# Autodesk Inventor assembly: Assembly_Cube_Lens_holder_v3
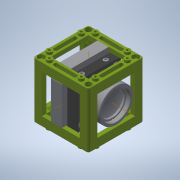
[picture p0: Inventor's stored thumbnail of the model, 180x180]
Saved by Autodesk Inventor 2022.3 (Build 263350000, 350)
## iProperties
Created: 2020-11-11
Part Number: Assembly_Cube_Lens_holder_v3
Document SubType Name: Assembly
Designer: marsikovabarbora
Author: marsikovabarbora
## Documents named in this file (5)
- G:\My Drive\ASP - M.Sc. Photonics\Practical Modules\MODULE 4 - Master Thesis\2.Experiments\Modules\8.Lens_Thorlabs_Module\Assembly_Cube_Thorlabs_Lens_Cage_v3.iam
- G:\My Drive\ASP - M.Sc. Photonics\Practical Modules\MODULE 4 - Master Thesis\2.Experiments\Modules\2.Base_Cube\Base_Cube_IM\Assembly_Cube_empty_IM_v3.iam
- G:\My Drive\ASP - M.Sc. Photonics\Practical Modules\MODULE 4 - Master Thesis\2.Experiments\Modules\8.Lens_Thorlabs_Module\00_Thorlabs_Cage_CP33_M.ipt
- G:\My Drive\ASP - M.Sc. Photonics\Practical Modules\MODULE 4 - Master Thesis\2.Experiments\Modules\8.Lens_Thorlabs_Module\20_Cube_Insert_Thorlabs_Pins.ipt
- G:\My Drive\ASP - M.Sc. Photonics\Practical Modules\MODULE 4 - Master Thesis\2.Experiments\Modules\8.Lens_Thorlabs_Module\00_THORLABS_AC254-050-A-ML-Step.ipt
## Components (4 placed, 4 different names)
1. Assembly_Cube_empty_IM_v3:1 [sub-assembly] — Mate:1, Mate:2, Mate:3, Passend:4, Passend:5
2. 00_Thorlabs_Cage_CP33_M:1 — Rigid:1
3. 20_Cube_Insert_Thorlabs_Pins:1 — Passend:4, Passend:5
4. 00_THORLABS_AC254-050-A-ML-Step:1 — Rigid:1
## Relationships (6: Mate 5, WeldJoint 1)
- Mate:1: Assembly_Cube_empty_IM_v3:1
- Mate:2: Assembly_Cube_empty_IM_v3:1
- Mate:3: Assembly_Cube_empty_IM_v3:1
- Passend:4 [Mate]: Assembly_Cube_empty_IM_v3:1 ↔ 20_Cube_Insert_Thorlabs_Pins:1
- Passend:5 [Mate]: Assembly_Cube_empty_IM_v3:1 ↔ 20_Cube_Insert_Thorlabs_Pins:1
- Rigid:1 [WeldJoint]: 00_Thorlabs_Cage_CP33_M:1 ↔ 00_THORLABS_AC254-050-A-ML-Step:1
